# Autodesk Inventor assembly: aos5
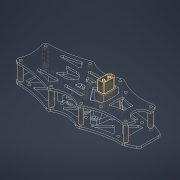
[picture p0: Inventor's stored thumbnail of the model, 180x180]
Saved by Autodesk Inventor 2022 (Build 260153000, 153)
## iProperties
Created: 2022-07-20
Part Number: aos5
Document SubType Name: Assembly
Designer: ancher
Author: ancher
## Documents named in this file (10)
- E:\RC\print_3d\aos5\aos5.iam
- E:\RC\print_3d\aos5\bottom_plate.ipt
- E:\RC\print_3d\aos5\top_plate.ipt
- E:\RC\print_3d\aos5\standoff.ipt
- E:\RC\print_3d\inventor\ContentCenterFiles\en-US\ISO 7380-1\ISO 7380-1 - M3 x 6.ipt
- E:\RC\print_3d\aos5\esc.iam
- E:\RC\print_3d\inventor\ContentCenterFiles\en-US\ISO 7380-1\ISO 7380-1 - M3 x 20.ipt
- E:\RC\print_3d\inventor\ContentCenterFiles\en-US\DIN 439-2\DIN 439 - M3 x 0.5.ipt
- E:\RC\print_3d\aos5\xt60_base.ipt
- E:\RC\print_3d\aos5\xt60h-m.ipt
## Components (29 placed, 9 different names)
1. bottom_plate:1 — Mate:1, Mate:2, Mate:3, Mate:4, Mate:5, Mate:6, Mate:7, Mate:8, Mate:9, Mate:11, Mate:12, Mate:13, Mate:14, Mate:15, Mate:16, Mate:17, Mate:18, Mate:19, Mate:21, Mate:23, Mate:25, Mate:27, Mate:29, Mate:31, Mate:33, Mate:35, Mate:36, Mate:37, Insert:1, Insert:2, Insert:3, Insert:4, Mate:39, Mate:41, Mate:43, Mate:45, Mate:48, Mate:49, Mate:50
2. top_plate:1 — Mate:1, Mate:2, Mate:47
3. esc:1 [sub-assembly] — Mate:36, Mate:37, Mate:46
4. xt60h-m:1 — Insert:5, Insert:6
5. xt60_base:1 — Mate:48, Mate:49, Mate:50, Insert:5, Insert:6
6. DIN 439-2 - replaced by DIN EN 24035/28675 M3:1 — Mate:38, Mate:39
7. DIN 439-2 - replaced by DIN EN 24035/28675 M3:2 — Mate:40, Mate:41
8. DIN 439-2 - replaced by DIN EN 24035/28675 M3:3 — Mate:42, Mate:43
9. DIN 439-2 - replaced by DIN EN 24035/28675 M3:4 — Mate:44, Mate:45, Mate:46
10. ISO 7380-1 M3 x 20:1 — Insert:1, Mate:40
11. ISO 7380-1 M3 x 20:2 — Insert:2, Mate:42
12. ISO 7380-1 M3 x 20:3 — Insert:3, Mate:38
13. ISO 7380-1 M3 x 20:4 — Insert:4, Mate:44
14. ISO 7380-1 M3 x 6:1 — Mate:20, Mate:21
15. ISO 7380-1 M3 x 6:2 — Mate:22, Mate:23
16. ISO 7380-1 M3 x 6:3 — Mate:24, Mate:25
17. ISO 7380-1 M3 x 6:4 — Mate:26, Mate:27
18. ISO 7380-1 M3 x 6:5 — Mate:28, Mate:29
19. ISO 7380-1 M3 x 6:6 — Mate:30, Mate:31
20. ISO 7380-1 M3 x 6:7 — Mate:32, Mate:33
21. ISO 7380-1 M3 x 6:8 — Mate:34, Mate:35
22. standoff:1 — Mate:3, Mate:11, Mate:22
23. standoff:2 — Mate:4, Mate:13, Mate:24
24. standoff:3 — Mate:5, Mate:17, Mate:26
25. standoff:4 — Mate:6, Mate:19, Mate:28
26. standoff:5 — Mate:7, Mate:18, Mate:30
27. standoff:6 — Mate:8, Mate:16, Mate:32
28. standoff:7 — Mate:9, Mate:15, Mate:34, Mate:47
29. standoff:8 — Mate:12, Mate:14, Mate:20
## Relationships (55: Mate 49, Insert 6)
- Mate:1: bottom_plate:1 ↔ top_plate:1
- Mate:2: bottom_plate:1 ↔ top_plate:1
- Mate:3: bottom_plate:1 ↔ standoff:1
- Mate:4: bottom_plate:1 ↔ standoff:2
- Mate:5: bottom_plate:1 ↔ standoff:3
- Mate:6: bottom_plate:1 ↔ standoff:4
- Mate:7: bottom_plate:1 ↔ standoff:5
- Mate:8: bottom_plate:1 ↔ standoff:6
- Mate:9: bottom_plate:1 ↔ standoff:7
- Mate:11: bottom_plate:1 ↔ standoff:1
- Mate:12: bottom_plate:1 ↔ standoff:8
- Mate:13: bottom_plate:1 ↔ standoff:2
- Mate:14: bottom_plate:1 ↔ standoff:8
- Mate:15: bottom_plate:1 ↔ standoff:7
- Mate:16: bottom_plate:1 ↔ standoff:6
- Mate:17: bottom_plate:1 ↔ standoff:3
- Mate:18: bottom_plate:1 ↔ standoff:5
- Mate:19: bottom_plate:1 ↔ standoff:4
- Mate:20: ISO 7380-1 M3 x 6:1 ↔ standoff:8
- Mate:21: bottom_plate:1 ↔ ISO 7380-1 M3 x 6:1
- Mate:22: ISO 7380-1 M3 x 6:2 ↔ standoff:1
- Mate:23: bottom_plate:1 ↔ ISO 7380-1 M3 x 6:2
- Mate:24: ISO 7380-1 M3 x 6:3 ↔ standoff:2
- Mate:25: bottom_plate:1 ↔ ISO 7380-1 M3 x 6:3
- Mate:26: ISO 7380-1 M3 x 6:4 ↔ standoff:3
- Mate:27: bottom_plate:1 ↔ ISO 7380-1 M3 x 6:4
- Mate:28: ISO 7380-1 M3 x 6:5 ↔ standoff:4
- Mate:29: bottom_plate:1 ↔ ISO 7380-1 M3 x 6:5
- Mate:30: ISO 7380-1 M3 x 6:6 ↔ standoff:5
- Mate:31: bottom_plate:1 ↔ ISO 7380-1 M3 x 6:6
- Mate:32: ISO 7380-1 M3 x 6:7 ↔ standoff:6
- Mate:33: bottom_plate:1 ↔ ISO 7380-1 M3 x 6:7
- Mate:34: ISO 7380-1 M3 x 6:8 ↔ standoff:7
- Mate:35: bottom_plate:1 ↔ ISO 7380-1 M3 x 6:8
- Mate:36: bottom_plate:1 ↔ esc:1
- Mate:37: bottom_plate:1 ↔ esc:1
- Insert:1: bottom_plate:1 ↔ ISO 7380-1 M3 x 20:1
- Insert:2: bottom_plate:1 ↔ ISO 7380-1 M3 x 20:2
- Insert:3: bottom_plate:1 ↔ ISO 7380-1 M3 x 20:3
- Insert:4: bottom_plate:1 ↔ ISO 7380-1 M3 x 20:4
- Mate:38: DIN 439-2 - replaced by DIN EN 24035/28675 M3:1 ↔ ISO 7380-1 M3 x 20:3
- Mate:39: bottom_plate:1 ↔ DIN 439-2 - replaced by DIN EN 24035/28675 M3:1
- Mate:40: DIN 439-2 - replaced by DIN EN 24035/28675 M3:2 ↔ ISO 7380-1 M3 x 20:1
- Mate:41: bottom_plate:1 ↔ DIN 439-2 - replaced by DIN EN 24035/28675 M3:2
- Mate:42: DIN 439-2 - replaced by DIN EN 24035/28675 M3:3 ↔ ISO 7380-1 M3 x 20:2
- Mate:43: bottom_plate:1 ↔ DIN 439-2 - replaced by DIN EN 24035/28675 M3:3
- Mate:44: DIN 439-2 - replaced by DIN EN 24035/28675 M3:4 ↔ ISO 7380-1 M3 x 20:4
- Mate:45: bottom_plate:1 ↔ DIN 439-2 - replaced by DIN EN 24035/28675 M3:4
- Mate:46: esc:1 ↔ DIN 439-2 - replaced by DIN EN 24035/28675 M3:4
- Mate:47: top_plate:1 ↔ standoff:7
- Mate:48: bottom_plate:1 ↔ xt60_base:1
- Mate:49: bottom_plate:1 ↔ xt60_base:1
- Mate:50: bottom_plate:1 ↔ xt60_base:1
- Insert:5: xt60h-m:1 ↔ xt60_base:1
- Insert:6: xt60h-m:1 ↔ xt60_base:1
